# Autodesk Inventor assembly: LeftSidePanelFull
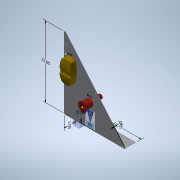
[picture p0: Inventor's stored thumbnail of the model, 180x180]
Saved by Autodesk Inventor 2021 (Build 250183000, 183)
## iProperties
Created: 2020-09-30
Part Number: LeftSidePanelFull
Document SubType Name: Assembly
Designer: Jonathan
Author: Jonathan
## Documents named in this file (6)
- D:\Scool\ECE 491\FullCarV2.2-20201122T225417Z-001\FullCarV2.2\SidePanels\LeftSidePanelFull.iam
- D:\Scool\ECE 491\Side_panels_11_1\LeftSidePanel2020.ipt
- D:\Scool\ECE 491\FullCarV2.2-20201122T225417Z-001\FullCarV2.2\SidePanels\SSOK.ipt
- D:\Scool\ECE 491\FullCarV2.2-20201122T225417Z-001\FullCarV2.2\SidePanels\estop.ipt
- D:\Scool\ECE 491\1470G1-IGS\1470G1.ipt
- D:\Scool\ECE 491\FullCarV2.2-20201122T225417Z-001\FullCarV2.2\SidePanels\9600K130_SBR RUBBER PUSH-IN GROMMET.ipt
## Components (5 placed, 5 different names)
1. LeftSidePanel2020:1 — Mate:1, Mate:2, Mate:3, Mate:4, Mate:5, Insert:1
2. SSOK:1 — Mate:3, Mate:4, Mate:5
3. estop:1 — Mate:1, Mate:2
4. 1470G1:1
5. 9600K130_SBR RUBBER PUSH-IN GROMMET:1 — Insert:1
## Relationships (6: Mate 5, Insert 1)
- Mate:1: LeftSidePanel2020:1 ↔ estop:1
- Mate:2: LeftSidePanel2020:1 ↔ estop:1
- Mate:3: LeftSidePanel2020:1 ↔ SSOK:1
- Mate:4: LeftSidePanel2020:1 ↔ SSOK:1
- Mate:5: LeftSidePanel2020:1 ↔ SSOK:1
- Insert:1: LeftSidePanel2020:1 ↔ 9600K130_SBR RUBBER PUSH-IN GROMMET:1
